# Autodesk Inventor assembly: Tape Measure Bracket Assembly V4
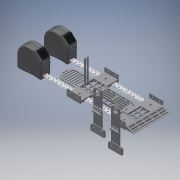
[picture p0: Inventor's stored thumbnail of the model, 180x180]
Saved by Autodesk Inventor 2019 (Build 230136000, 136)
## iProperties
Created: 2018-11-08
Part Number: Tape Measure Bracket Assembly V4
Document SubType Name: Assembly
Designer: Ashley
Author: Ashley
## Documents named in this file (5)
- C:\Users\Ashley\Desktop\repositories\design\inventor\2018-2019\Tape Measure Braket\Version Four\Tape Measure Bracket Assembly V4.iam
- C:\Users\Ashley\Desktop\repositories\design\inventor\2018-2019\Tape Measure Braket\Version Four\Bracket Bottom V4.ipt
- C:\Users\Ashley\Desktop\repositories\design\inventor\2018-2019\Tape Measure Braket\Tape Measure\Tape Measure Edited.iam
- C:\Users\Ashley\Desktop\repositories\design\inventor\2018-2019\Tape Measure Braket\Version Four\Side V4.ipt
- C:\Users\Ashley\Desktop\repositories\design\inventor\2018-2019\Tape Measure Braket\Version Two\Braket Top V2.ipt
## Components (10 placed, 8 different names)
1. Bracket Bottom — Mate:4, Mate:5
2. Tape Measure Right [sub-assembly]
3. Tape Measure Left [sub-assembly]
4. Top Back Right — Mate:5
5. Top Back Left — Mate:4
6. Top Front Right
7. Top Front Left
8. Side V4:1
9. Side V4:2
10. Side V4:3
## Relationships (2: Mate 2)
- Mate:4: Bracket Bottom ↔ Top Back Left
- Mate:5: Bracket Bottom ↔ Top Back Right
